# Autodesk Inventor assembly: first_floor_simplified
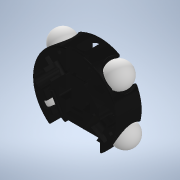
[picture p0: Inventor's stored thumbnail of the model, 180x180]
Saved by Autodesk Inventor 2021 (Build 250183000, 183)
## iProperties
Created: 2022-08-10
Part Number: first_floor_simplified
Document SubType Name: Assembly
Designer: victo
Title: C:\Users\victo\Documents\MATLAB\CAD\Inventor\first_floor\first_floor_simplified.stp
Author: victo
Sending System: Autodesk Inventor 2023
Preprocessor: ST-DEVELOPER v19
## Documents named in this file (3)
- C:\Users\victo\Documents\MATLAB\CAD\Inventor\first_floor\first_floor_simplified.iam
- C:\Users\victo\Documents\MATLAB\CAD\Inventor\first_floor\Base_RoboCIn_simplified.ipt
- C:\Users\victo\Documents\MATLAB\CAD\Inventor\first_floor\wheel_simplified.ipt
## Components (5 placed, 2 different names)
1. Base_RoboCIn_simplified:1 — Mate:1, Mate:2, Mate:3, Mate:4
2. wheel_simplified:1 — Mate:2
3. wheel_simplified:2 — Mate:3
4. wheel_simplified:3 — Mate:1
5. wheel_simplified:4 — Mate:4
## Relationships (4: Mate 4)
- Mate:1: Base_RoboCIn_simplified:1 ↔ wheel_simplified:3
- Mate:2: Base_RoboCIn_simplified:1 ↔ wheel_simplified:1
- Mate:3: Base_RoboCIn_simplified:1 ↔ wheel_simplified:2
- Mate:4: Base_RoboCIn_simplified:1 ↔ wheel_simplified:4
